# Autodesk Inventor assembly: curved-+_plates_MIR
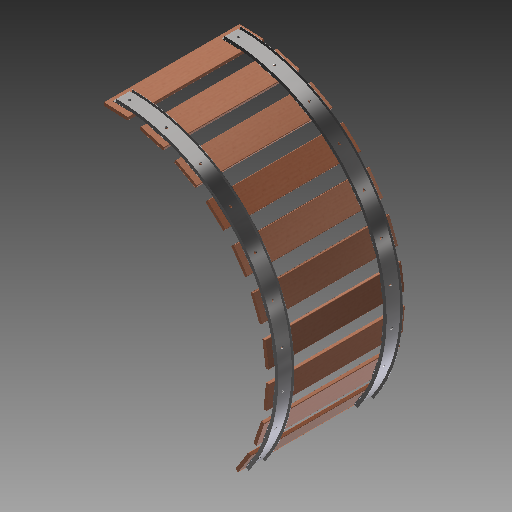
[picture p0: Inventor's stored thumbnail of the model, 512x512]
Saved by Autodesk Inventor 2019 (Build 230136000, 136)
## iProperties
Created: 2019-02-24
Part Number: curved-+_plates_MIR
Document SubType Name: Assembly
Designer: gaincarlo
Author: gaincarlo
## Documents named in this file (3)
- D:\Giancarlo Bacchio\Documenti\00 - Progetti\30-Inventor\LaPanca\curved-+_plates_MIR.iam
- D:\Giancarlo Bacchio\Documenti\00 - Progetti\30-Inventor\LaPanca\support2_MIR.ipt
- D:\Giancarlo Bacchio\Documenti\00 - Progetti\30-Inventor\LaPanca\doga_short_MIR.ipt
## Components (12 placed, 2 different names)
1. support2_MIR:1 — Mate:3, Mate:1
2. support2_MIR:2 — Mate:2
3. doga_short_MIR:1 — Mate:3, Mate:1, Mate:2
4. doga_short_MIR:2
5. doga_short_MIR:3
6. doga_short_MIR:4
7. doga_short_MIR:5
8. doga_short_MIR:6
9. doga_short_MIR:7
10. doga_short_MIR:8
11. doga_short_MIR:9
12. doga_short_MIR:10
## Component patterns: (10 elements, first: doga_short_MIR:1)
## Relationships (3: Mate 3)
- Mate:3: support2_MIR:1 ↔ doga_short_MIR:1
- Mate:1: support2_MIR:1 ↔ doga_short_MIR:1
- Mate:2: support2_MIR:2 ↔ doga_short_MIR:1
